# Autodesk Inventor assembly: Assembly2
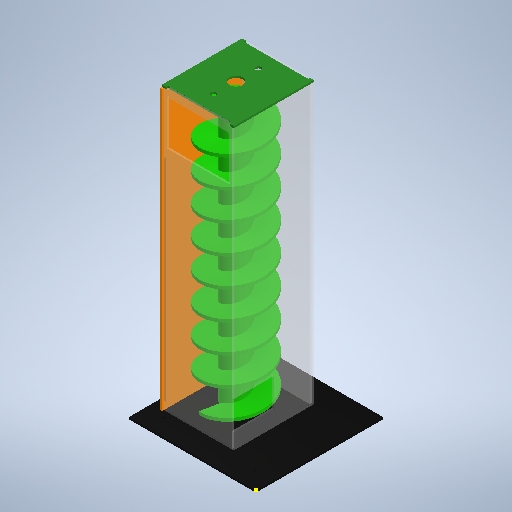
[picture p0: Inventor's stored thumbnail of the model, 512x512]
Saved by Autodesk Inventor 2025.4 (Build 294407000, 407)
## iProperties
Created: 2026-04-06
Part Number: Assembly2
Document SubType Name: Assembly
Designer: abdo2
Author: abdo2
## Documents named in this file (8)
- F:\ASU Engineering\Year.2 ( 25-26 )\Spring\Basics Of Mechatronics\Project\Mechanisms\Lifting Mechanism\Assembly2.iam
- F:\ASU Engineering\Year.2 ( 25-26 )\Spring\Basics Of Mechatronics\Project\Mechanisms\Lifting Mechanism\Part 1 base.ipt
- F:\ASU Engineering\Year.2 ( 25-26 )\Spring\Basics Of Mechatronics\Project\Mechanisms\Lifting Mechanism\lifting cover.ipt
- F:\ASU Engineering\Year.2 ( 25-26 )\Spring\Basics Of Mechatronics\Project\Mechanisms\Lifting Mechanism\lifting cover 2.ipt
- F:\ASU Engineering\Year.2 ( 25-26 )\Spring\Basics Of Mechatronics\Project\Mechanisms\Lifting Mechanism\Lifting mechanism.ipt
- F:\ASU Engineering\Year.2 ( 25-26 )\Spring\Basics Of Mechatronics\Project\Mechanisms\Lifting Mechanism\ackleryk.ipt
- F:\ASU Engineering\Year.2 ( 25-26 )\Spring\Basics Of Mechatronics\Project\Mechanisms\Lifting Mechanism\Lift cover of lifting.ipt
- F:\ASU Engineering\Year.2 ( 25-26 )\Spring\Basics Of Mechatronics\Project\Mechanisms\Lifting Mechanism\upper support.ipt
## Components (7 placed, 7 different names)
1. Part 1 base:1 — Mate:16, Mate:17, Mate:18, Mate:25, Mate:26, Mate:55, Mate:91, Mate:92, Mate:93
2. lifting cover:2 — Mate:16, Mate:17, Mate:18, Mate:19, Mate:20, Mate:21, Mate:56, Flush:2
3. lifting cover 2:1 — Mate:19, Mate:20, Mate:21, Mate:96
4. Lifting mechanism:1 — Mate:25, Mate:26, Mate:98
5. ackleryk:1 — Mate:55, Mate:56, Flush:2, Flush:3
6. Lift cover of lifting:1 — Mate:91, Mate:92, Mate:93
7. upper support:1 — Mate:96, Mate:98, Flush:3
## Relationships (17: Mate 15, Flush 2)
- Mate:16: Part 1 base:1 ↔ lifting cover:2
- Mate:17: Part 1 base:1 ↔ lifting cover:2
- Mate:18: Part 1 base:1 ↔ lifting cover:2
- Mate:19: lifting cover:2 ↔ lifting cover 2:1
- Mate:20: lifting cover:2 ↔ lifting cover 2:1
- Mate:21: lifting cover:2 ↔ lifting cover 2:1
- Mate:25: Part 1 base:1 ↔ Lifting mechanism:1
- Mate:26 (7 mm): Part 1 base:1 ↔ Lifting mechanism:1
- Mate:55: Part 1 base:1 ↔ ackleryk:1
- Mate:56: lifting cover:2 ↔ ackleryk:1
- Mate:91: Part 1 base:1 ↔ Lift cover of lifting:1
- Mate:92: Part 1 base:1 ↔ Lift cover of lifting:1
- Mate:93: Part 1 base:1 ↔ Lift cover of lifting:1
- Flush:2: lifting cover:2 ↔ ackleryk:1
- Mate:96: lifting cover 2:1 ↔ upper support:1
- Mate:98: Lifting mechanism:1 ↔ upper support:1
- Flush:3: ackleryk:1 ↔ upper support:1
